# Autodesk Inventor assembly: Chassis-SubAssem01
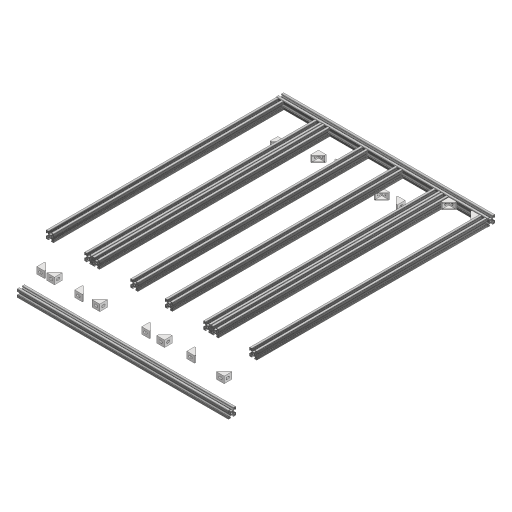
[picture p0: Inventor's stored thumbnail of the model, 512x512]
Saved by Autodesk Inventor 2024 (Build 280153000, 153)
## iProperties
Created: 2023-10-26
Part Number: Chassis-SubAssem01
Document SubType Name: Assembly
Designer: david
Author: david
## Documents named in this file (5)
- C:\Autodesk\ChalkBot Github\ChalkbotMechanical\Chalkbot1.0\Chassis\V1\Chassis-SubAssem01.iam
- C:\Autodesk\ChalkBot Github\ChalkbotMechanical\Chalkbot1.0\Chassis\V1\20x20 Channel\20x20 Channel-550.ipt
- C:\Autodesk\ChalkBot Github\ChalkbotMechanical\Chalkbot1.0\Chassis\V1\20x20 Channel.ipt
- C:\Autodesk\ChalkBot Github\ChalkbotMechanical\Chalkbot1.0\Chassis\V1\20x20 Channel\20x20 Channel-600.ipt
- C:\Autodesk\ChalkBot Github\ChalkbotMechanical\Chalkbot1.0\Chassis\V1\20x20 90 Gusset.ipt
## Components (26 placed, 3 different names)
1. 20x20 Channel-550:1
2. 20x20 Channel-550:2 — Mate:1, Flush:1, Mate:3, Flush:3, Flush:4, Mate:5, Flush:5, Mate:7, Flush:6, Mate:9, Mate:11, Flush:7, Flush:9, Mate:12, Flush:10, Mate:15
3. 20x20 Channel-600:3 — Mate:13, Flush:10, Mate:15
4. 20x20 Channel-600:4 — Rigid:2, Flush:9, Mate:12, Mate:14
5. 20x20 Channel-600:5 — Rigid:2, Mate:13
6. 20x20 Channel-600:6 — Mate:10, Mate:11, Flush:7, Mate:14
7. 20x20 Channel-600:7 — Mate:8, Flush:6, Mate:9, Mate:10
8. 20x20 Channel-600:8 — Rigid:1, Flush:4, Mate:8
9. 20x20 Channel-600:9 — Rigid:1, Mate:4, Mate:5, Mate:6
10. 20x20 Channel-600:10 — Mate:2, Flush:2, Mate:3, Flush:3, Mate:4
11. 20x20 90 Gusset:1
12. 20x20 90 Gusset:2
13. 20x20 90 Gusset:3
14. 20x20 90 Gusset:4
15. 20x20 90 Gusset:5
16. 20x20 90 Gusset:6 — Flush:5, Mate:6, Mate:7
17. 20x20 90 Gusset:7
18. 20x20 90 Gusset:8
19. 20x20 90 Gusset:9 — Mate:1, Flush:1, Mate:2, Flush:2
20. 20x20 90 Gusset:10
21. 20x20 90 Gusset:11
22. 20x20 90 Gusset:12
23. 20x20 90 Gusset:13
24. 20x20 90 Gusset:14
25. 20x20 90 Gusset:15
26. 20x20 90 Gusset:16
## Relationships (26: Mate 15, Flush 9, WeldJoint 2)
- Rigid:1 [WeldJoint]: 20x20 Channel-600:8 ↔ 20x20 Channel-600:9
- Rigid:2 [WeldJoint]: 20x20 Channel-600:4 ↔ 20x20 Channel-600:5
- Mate:1: 20x20 Channel-550:2 ↔ 20x20 90 Gusset:9
- Flush:1 (1.5 mm): 20x20 Channel-550:2 ↔ 20x20 90 Gusset:9
- Mate:2: 20x20 Channel-600:10 ↔ 20x20 90 Gusset:9
- Flush:2 (1.5 mm): 20x20 Channel-600:10 ↔ 20x20 90 Gusset:9
- Mate:3: 20x20 Channel-550:2 ↔ 20x20 Channel-600:10
- Flush:3: 20x20 Channel-550:2 ↔ 20x20 Channel-600:10
- Mate:4 (80 mm): 20x20 Channel-600:9 ↔ 20x20 Channel-600:10
- Flush:4: 20x20 Channel-550:2 ↔ 20x20 Channel-600:8
- Mate:5: 20x20 Channel-550:2 ↔ 20x20 Channel-600:9
- Flush:5 (1.5 mm): 20x20 Channel-550:2 ↔ 20x20 90 Gusset:6
- Mate:6: 20x20 Channel-600:9 ↔ 20x20 90 Gusset:6
- Mate:7: 20x20 Channel-550:2 ↔ 20x20 90 Gusset:6
- Mate:8 (80 mm): 20x20 Channel-600:7 ↔ 20x20 Channel-600:8
- Flush:6: 20x20 Channel-550:2 ↔ 20x20 Channel-600:7
- Mate:9: 20x20 Channel-550:2 ↔ 20x20 Channel-600:7
- Mate:10 (70 mm): 20x20 Channel-600:6 ↔ 20x20 Channel-600:7
- Mate:11: 20x20 Channel-550:2 ↔ 20x20 Channel-600:6
- Flush:7: 20x20 Channel-550:2 ↔ 20x20 Channel-600:6
- Flush:9: 20x20 Channel-550:2 ↔ 20x20 Channel-600:4
- Mate:12: 20x20 Channel-550:2 ↔ 20x20 Channel-600:4
- Mate:13 (80 mm): 20x20 Channel-600:3 ↔ 20x20 Channel-600:5
- Mate:14 (80 mm): 20x20 Channel-600:4 ↔ 20x20 Channel-600:6
- Flush:10: 20x20 Channel-550:2 ↔ 20x20 Channel-600:3
- Mate:15: 20x20 Channel-550:2 ↔ 20x20 Channel-600:3
